# Autodesk Inventor assembly: 000.005 -  Манипулятор
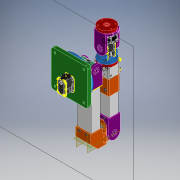
[picture p0: Inventor's stored thumbnail of the model, 180x180]
Saved by Autodesk Inventor 2022 (Build 260153000, 153)
## iProperties
Created: 2022-11-17
Part Number: 000.005 -  Манипулятор
Document SubType Name: Assembly
Designer: Petrov Ivan
Mass: 2549.27 g
Surface Area: 6811.79 cm^2
Volume: 2245.98 cm^3
Density: 1.13504 g/cm^3
Author: Petrov Ivan
## Documents named in this file (8)
- C:\Users\Ivan Petrov\Documents\GitHub\OmniBot\design\000.005 -  Манипулятор.iam
- C:\Users\Ivan Petrov\Documents\GitHub\OmniBot\design\000.005.001 - Поворотный стол.iam
- C:\Users\Ivan Petrov\Documents\GitHub\OmniBot\design\000.005.002 - Плечо СБ.iam
- C:\Users\Ivan Petrov\Documents\GitHub\OmniBot\design\000.005.003 - Локоть СБ.iam
- C:\Users\Ivan Petrov\Documents\GitHub\OmniBot\design\Content Center Files\R2022\ru-RU\ISO 4762(1)\DIN EN ISO 4762 - M4 x 16.ipt
- C:\Users\Ivan Petrov\Documents\GitHub\OmniBot\design\000.005.004 - Поворот сгиба кисти СБ.iam
- C:\Users\Ivan Petrov\Documents\GitHub\OmniBot\design\000.005.005 - Сгиб кисти.iam
- 000.005.005 - Сгиб кисти СБ.iam
## Components (9 placed, 6 different names)
1. 000.005.001 - Поворотный стол СБ:1 [sub-assembly] — Совмещение:1, Совмещение:2, Совмещение:3, Угол:1, Угол:2
2. 000.005.002 - Плечо СБ:1 [sub-assembly] — Совмещение:1, Совмещение:2, Совмещение:3, Вставка:1, Вставка:2, Вставка:3, Вставка:4, Угол:1, Совмещение:4, Совмещение:5, Совмещение:6, Угол:2, Угол:3
3. 000.005.003 - Локоть СБ:1 [sub-assembly] — Совмещение:4, Совмещение:5, Совмещение:6, Угол:3, Угол:4, Угол:5, Совмещение:7, Совмещение:8, Совмещение:9
4. DIN EN ISO 4762 M4 x 16:1 — Вставка:1
5. DIN EN ISO 4762 M4 x 16:2 — Вставка:2
6. DIN EN ISO 4762 M4 x 16:3 — Вставка:3
7. DIN EN ISO 4762 M4 x 16:4 — Вставка:4
8. 000.005.004 - Поворот сгиба кисти СБ:1 [sub-assembly] — Совмещение:7, Совмещение:8, Совмещение:9, Совмещение:10, Совмещение:11, Совмещение:12
9. 000.005.005 - Сгиб кисти СБ:1 [sub-assembly] — Совмещение:10, Совмещение:11, Совмещение:12
## Relationships (21: Mate 12, Angle 5, Insert 4)
- Совмещение:1 [Mate]: 000.005.001 - Поворотный стол СБ:1 ↔ 000.005.002 - Плечо СБ:1
- Совмещение:2 [Mate]: 000.005.001 - Поворотный стол СБ:1 ↔ 000.005.002 - Плечо СБ:1
- Совмещение:3 [Mate]: 000.005.001 - Поворотный стол СБ:1 ↔ 000.005.002 - Плечо СБ:1
- Вставка:1 [Insert]: 000.005.002 - Плечо СБ:1 ↔ DIN EN ISO 4762 M4 x 16:1
- Вставка:2 [Insert]: 000.005.002 - Плечо СБ:1 ↔ DIN EN ISO 4762 M4 x 16:2
- Вставка:3 [Insert]: 000.005.002 - Плечо СБ:1 ↔ DIN EN ISO 4762 M4 x 16:3
- Вставка:4 [Insert]: 000.005.002 - Плечо СБ:1 ↔ DIN EN ISO 4762 M4 x 16:4
- Угол:1 [Angle] (180 deg): 000.005.001 - Поворотный стол СБ:1 ↔ 000.005.002 - Плечо СБ:1
- Совмещение:4 [Mate]: 000.005.002 - Плечо СБ:1 ↔ 000.005.003 - Локоть СБ:1
- Совмещение:5 [Mate] (0.25 mm): 000.005.002 - Плечо СБ:1 ↔ 000.005.003 - Локоть СБ:1
- Совмещение:6 [Mate] (0.25 mm): 000.005.002 - Плечо СБ:1 ↔ 000.005.003 - Локоть СБ:1
- Угол:2 [Angle] (0 deg): 000.005.001 - Поворотный стол СБ:1 ↔ 000.005.002 - Плечо СБ:1
- Угол:3 [Angle] (0 deg): 000.005.002 - Плечо СБ:1 ↔ 000.005.003 - Локоть СБ:1
- Угол:4 [Angle] (0 deg): 000.005.003 - Локоть СБ:1
- Угол:5 [Angle] (0 deg): 000.005.003 - Локоть СБ:1
- Совмещение:7 [Mate]: 000.005.003 - Локоть СБ:1 ↔ 000.005.004 - Поворот сгиба кисти СБ:1
- Совмещение:8 [Mate]: 000.005.003 - Локоть СБ:1 ↔ 000.005.004 - Поворот сгиба кисти СБ:1
- Совмещение:9 [Mate]: 000.005.003 - Локоть СБ:1 ↔ 000.005.004 - Поворот сгиба кисти СБ:1
- Совмещение:10 [Mate]: 000.005.004 - Поворот сгиба кисти СБ:1 ↔ 000.005.005 - Сгиб кисти СБ:1
- Совмещение:11 [Mate]: 000.005.004 - Поворот сгиба кисти СБ:1 ↔ 000.005.005 - Сгиб кисти СБ:1
- Совмещение:12 [Mate]: 000.005.004 - Поворот сгиба кисти СБ:1 ↔ 000.005.005 - Сгиб кисти СБ:1
